# Autodesk Inventor assembly: робот - сборка фулл
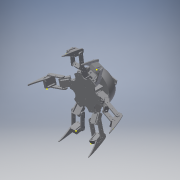
[picture p0: Inventor's stored thumbnail of the model, 180x180]
Saved by Autodesk Inventor 2019 (Build 230136000, 136)
## iProperties
Created: 2019-09-07
Part Number: робот - сборка фулл
Material: Типовые
Document SubType Name: Assembly
Designer: Iliga
Author: Iliga
## Documents named in this file (12)
- C:\Users\UlyaKZ\Desktop\робот3\робот - сборка фулл.iam
- C:\Users\UlyaKZ\Desktop\робот3\тело.ipt
- C:\Users\UlyaKZ\Desktop\робот3\левая лапа - сборка.iam
- C:\Users\UlyaKZ\Desktop\робот3\правая лапа - сборка.iam
- C:\Users\UlyaKZ\Desktop\робот3\крепление2.ipt
- C:\Users\UlyaKZ\Desktop\робот3\крепление-стенки.ipt
- C:\Users\UlyaKZ\Desktop\робот3\хребет2.ipt
- C:\Users\UlyaKZ\Desktop\робот3\полочка.ipt
- C:\Users\UlyaKZ\Desktop\робот3\мотор.ipt
- C:\Users\UlyaKZ\Desktop\робот3\креплениекамеры.ipt
- C:\Users\UlyaKZ\Desktop\робот3\креплениедлякамерыниз.ipt
- C:\Users\UlyaKZ\Desktop\робот3\креплениедлякамерыверх.ipt
## Components (16 placed, 11 different names)
1. лапа:1 [sub-assembly] — Совмещение:92, Совмещение:97
2. лапа:2 [sub-assembly] — Совмещение:89, Совмещение:91
3. правая лапа - сборка:1 [sub-assembly] — Совмещение:95, Совмещение:100
4. правая лапа - сборка:2 [sub-assembly] — Совмещение:93, Совмещение:98
5. правая лапа - сборка:3 [sub-assembly] — Совмещение:94, Совмещение:99
6. лапа:3 [sub-assembly] — Совмещение:90, Совмещение:96
7. крепление-стенки:1 — Совмещение:51, Совмещение:86, Совмещение:87, Совмещение:88, Совмещение:104, Совмещение:105
8. крепление2:1 — Совмещение:86, Совмещение:87, Совмещение:88, Совмещение:89, Совмещение:90, Совмещение:91, Совмещение:92, Совмещение:93, Совмещение:94, Совмещение:95, Совмещение:96, Совмещение:97, Совмещение:98, Совмещение:99, Совмещение:100
9. тело основа:1 — Совмещение:49, Совмещение:51, Заподлицо:1, Совмещение:101, Совмещение:102, Совмещение:103, Совмещение:104, Совмещение:105, Касательность:1, Совмещение:107, Совмещение:108, Совмещение:109, Совмещение:110, Совмещение:112
10. тело основа:2 — Совмещение:49, Заподлицо:1, Касательность:1
11. полочка:1 — Совмещение:101, Совмещение:102, Совмещение:103
12. хребет2:1 — Совмещение:107, Совмещение:108
13. мотор:1 — Совмещение:109, Совмещение:110, Совмещение:111
14. креплениекамеры:1 — Совмещение:111, Совмещение:112, Совмещение:113, Совмещение:114
15. креплениедлякамерыниз:1 — Совмещение:113, Совмещение:114, Совмещение:115, Совмещение:116, Совмещение:117
16. креплениедлякамерыверх:1 — Совмещение:115, Совмещение:116, Совмещение:117
## Relationships (35: Mate 33, Flush 1, Tangent 1)
- Совмещение:49 [Mate]: тело основа:1 ↔ тело основа:2
- Совмещение:51 [Mate]: крепление-стенки:1 ↔ тело основа:1
- Заподлицо:1 [Flush]: тело основа:1 ↔ тело основа:2
- Совмещение:86 [Mate]: крепление-стенки:1 ↔ крепление2:1
- Совмещение:87 [Mate]: крепление-стенки:1 ↔ крепление2:1
- Совмещение:88 [Mate]: крепление-стенки:1 ↔ крепление2:1
- Совмещение:89 [Mate]: лапа:2 ↔ крепление2:1
- Совмещение:90 [Mate]: лапа:3 ↔ крепление2:1
- Совмещение:91 [Mate]: лапа:2 ↔ крепление2:1
- Совмещение:92 [Mate]: лапа:1 ↔ крепление2:1
- Совмещение:93 [Mate]: правая лапа - сборка:2 ↔ крепление2:1
- Совмещение:94 [Mate]: правая лапа - сборка:3 ↔ крепление2:1
- Совмещение:95 [Mate]: правая лапа - сборка:1 ↔ крепление2:1
- Совмещение:96 [Mate]: лапа:3 ↔ крепление2:1
- Совмещение:97 [Mate]: лапа:1 ↔ крепление2:1
- Совмещение:98 [Mate]: правая лапа - сборка:2 ↔ крепление2:1
- Совмещение:99 [Mate]: правая лапа - сборка:3 ↔ крепление2:1
- Совмещение:100 [Mate]: правая лапа - сборка:1 ↔ крепление2:1
- Совмещение:101 [Mate]: тело основа:1 ↔ полочка:1
- Совмещение:102 [Mate]: тело основа:1 ↔ полочка:1
- Совмещение:103 [Mate] (84.7 mm): тело основа:1 ↔ полочка:1
- Совмещение:104 [Mate]: крепление-стенки:1 ↔ тело основа:1
- Совмещение:105 [Mate]: крепление-стенки:1 ↔ тело основа:1
- Касательность:1 [Tangent]: тело основа:1 ↔ тело основа:2
- Совмещение:107 [Mate]: тело основа:1 ↔ хребет2:1
- Совмещение:108 [Mate]: тело основа:1 ↔ хребет2:1
- Совмещение:109 [Mate]: тело основа:1 ↔ мотор:1
- Совмещение:110 [Mate]: тело основа:1 ↔ мотор:1
- Совмещение:111 [Mate]: мотор:1 ↔ креплениекамеры:1
- Совмещение:112 [Mate]: тело основа:1 ↔ креплениекамеры:1
- Совмещение:113 [Mate]: креплениекамеры:1 ↔ креплениедлякамерыниз:1
- Совмещение:114 [Mate]: креплениекамеры:1 ↔ креплениедлякамерыниз:1
- Совмещение:115 [Mate]: креплениедлякамерыниз:1 ↔ креплениедлякамерыверх:1
- Совмещение:116 [Mate]: креплениедлякамерыниз:1 ↔ креплениедлякамерыверх:1
- Совмещение:117 [Mate]: креплениедлякамерыниз:1 ↔ креплениедлякамерыверх:1
